# Autodesk Inventor assembly: big pulley
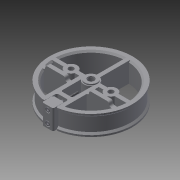
[picture p0: Inventor's stored thumbnail of the model, 180x180]
Saved by Autodesk Inventor 2013 (Build 170138000, 138)
## iProperties
Created: 2013-10-14
Part Number: big pulley
Document SubType Name: Assembly
Designer: employee
Author: employee
## Documents named in this file (6)
- C:\Users\employee\Desktop\new wally\big pulley.iam
- C:\Users\employee\Desktop\new wally\big pulley.ipt
- C:\Users\employee\Desktop\new wally\m3 nut.ipt
- C:\Users\employee\Desktop\new wally\string tensioner.ipt
- C:\Users\employee\Desktop\new wally\M3x35.ipt
- C:\Users\employee\Desktop\new wally\washer.ipt
## Components (7 placed, 5 different names)
1. big pulley:1 — Insert:1, Insert:2, Angle:1, Angle:2, Insert:3, Mate:1, Insert:6
2. Hex Nut Metric M3 x 0.5:1 — Insert:2, Angle:2
3. Hex Nut Metric M3 x 0.5:2 — Insert:1, Angle:1
4. string tensioner:1 — Insert:3, Mate:1, Insert:4, Insert:5
5. M3x35:1 — Insert:5
6. M3x35:2 — Insert:4
7. washer:1 — Insert:6
## Relationships (9: Insert 6, Angle 2, Mate 1)
- Insert:1: big pulley:1 ↔ Hex Nut Metric M3 x 0.5:2
- Insert:2: big pulley:1 ↔ Hex Nut Metric M3 x 0.5:1
- Angle:1 (0 deg): big pulley:1 ↔ Hex Nut Metric M3 x 0.5:2
- Angle:2 (0 deg): big pulley:1 ↔ Hex Nut Metric M3 x 0.5:1
- Insert:3 (5 mm): big pulley:1 ↔ string tensioner:1
- Mate:1: big pulley:1 ↔ string tensioner:1
- Insert:4: string tensioner:1 ↔ M3x35:2
- Insert:5: string tensioner:1 ↔ M3x35:1
- Insert:6: big pulley:1 ↔ washer:1
